# Autodesk Inventor assembly: Arduino UNO R3 screw Shield v2 Right
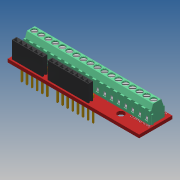
[picture p0: Inventor's stored thumbnail of the model, 180x180]
Saved by Autodesk Inventor 2017 SP1 (Build 210196100, 196)
## iProperties
Created: 2022-11-04
Part Number: Arduino UNO R3 screw Shield v2 Right
Document SubType Name: Assembly
Designer: Antonio
Author: Antonio
## Documents named in this file (7)
- C:\Users\Antonio\Documents\Inventor\Secador v2\Arduino UNO R3 screw shield v2\Arduino UNO R3 screw Shield v2 Right.iam
- C:\Users\Antonio\Documents\Inventor\Secador v2\DG381-3.5-06P-14-00AH.ipt
- C:\Users\Antonio\Documents\Inventor\Secador v2\Pin Header 1x6 TH Pitch 2.54mm.ipt
- C:\Users\Antonio\Documents\Inventor\Secador v2\Pin Header 1x8 TH Pitch 2.54mm.ipt
- C:\Users\Antonio\Documents\Inventor\Secador v2\HEMBRA 6 PINESB.ipt
- C:\Users\Antonio\Documents\Inventor\Secador v2\HEMBRA 8 PINESB.ipt
- C:\Users\Antonio\Documents\Inventor\Secador v2\Arduino UNO R3 screw shield v2\Arduino UNO R3 screw shield v2 board Right.ipt
## Components (8 placed, 6 different names)
1. DG381-3.5-06P-14-00AH:1 — Coincidencia:2, Nivelación:3, Nivelación:4, Coincidencia:10, Nivelación:10, Nivelación:11
2. DG381-3.5-06P-14-00AH:2 — Coincidencia:2, Nivelación:3, Nivelación:4, Coincidencia:3, Nivelación:5, Nivelación:6
3. DG381-3.5-06P-14-00AH:3 — Coincidencia:3, Nivelación:5, Nivelación:6
4. Pin Header 1x6 TH Pitch 2.54mm:1 — Coincidencia:6, Nivelación:12, Nivelación:13
5. Pin Header 1x8 TH Pitch 2.54mm:1 — Coincidencia:6, Nivelación:13
6. HEMBRA 6 PINESB:1 — Nivelación:14, Nivelación:15, Nivelación:16, Coincidencia:11, Nivelación:17
7. HEMBRA 8 PINESB:1 — Nivelación:16, Coincidencia:11, Nivelación:17
8. Arduino UNO R3 screw shield v2 board Right:1 — Coincidencia:10, Nivelación:10, Nivelación:11, Nivelación:12, Nivelación:14, Nivelación:15
## Relationships (17: Flush 12, Mate 5)
- Coincidencia:2 [Mate]: DG381-3.5-06P-14-00AH:1 ↔ DG381-3.5-06P-14-00AH:2
- Nivelación:3 [Flush]: DG381-3.5-06P-14-00AH:1 ↔ DG381-3.5-06P-14-00AH:2
- Nivelación:4 [Flush]: DG381-3.5-06P-14-00AH:1 ↔ DG381-3.5-06P-14-00AH:2
- Coincidencia:3 [Mate]: DG381-3.5-06P-14-00AH:2 ↔ DG381-3.5-06P-14-00AH:3
- Nivelación:5 [Flush]: DG381-3.5-06P-14-00AH:2 ↔ DG381-3.5-06P-14-00AH:3
- Nivelación:6 [Flush]: DG381-3.5-06P-14-00AH:2 ↔ DG381-3.5-06P-14-00AH:3
- Coincidencia:6 [Mate] (2.54 mm): Pin Header 1x6 TH Pitch 2.54mm:1 ↔ Pin Header 1x8 TH Pitch 2.54mm:1
- Coincidencia:10 [Mate]: DG381-3.5-06P-14-00AH:1 ↔ Arduino UNO R3 screw shield v2 board Right:1
- Nivelación:10 [Flush] (-1.25 mm): DG381-3.5-06P-14-00AH:1 ↔ Arduino UNO R3 screw shield v2 board Right:1
- Nivelación:11 [Flush] (-2.51 mm): DG381-3.5-06P-14-00AH:1 ↔ Arduino UNO R3 screw shield v2 board Right:1
- Nivelación:12 [Flush] (1.3 mm): Pin Header 1x6 TH Pitch 2.54mm:1 ↔ Arduino UNO R3 screw shield v2 board Right:1
- Nivelación:13 [Flush]: Pin Header 1x6 TH Pitch 2.54mm:1 ↔ Pin Header 1x8 TH Pitch 2.54mm:1
- Nivelación:14 [Flush] (1.29 mm): HEMBRA 6 PINESB:1 ↔ Arduino UNO R3 screw shield v2 board Right:1
- Nivelación:15 [Flush] (0.75 mm): HEMBRA 6 PINESB:1 ↔ Arduino UNO R3 screw shield v2 board Right:1
- Nivelación:16 [Flush]: HEMBRA 6 PINESB:1 ↔ HEMBRA 8 PINESB:1
- Coincidencia:11 [Mate] (2.54 mm): HEMBRA 6 PINESB:1 ↔ HEMBRA 8 PINESB:1
- Nivelación:17 [Flush]: HEMBRA 6 PINESB:1 ↔ HEMBRA 8 PINESB:1
